# Autodesk Inventor assembly: ArmSquare
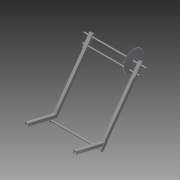
[picture p0: Inventor's stored thumbnail of the model, 180x180]
Saved by Autodesk Inventor 2013 (Build 170138000, 138)
## iProperties
Created: 2014-01-20
Part Number: ArmSquare
Document SubType Name: Assembly
Designer: RobertB
Author: RobertB
## Documents named in this file (10)
- E:\Robotics\FRC\2014\CAD\Robot\Catapult\Arm\ArmSquare.iam
- E:\Robotics\FRC\2014\CAD\Robot\Catapult\Arm\BarHolder.ipt
- E:\Robotics\FRC\2014\CAD\Robot\Catapult\Arm\CatapultAxle.ipt
- E:\Robotics\FRC\2014\CAD\Robot\Catapult\Arm\CatapultSprocket.ipt
- E:\Robotics\FRC\2014\CAD\Robot\Catapult\Arm\CatapultAxleSupportSquare.ipt
- E:\Robotics\FRC\2014\CAD\Robot\Catapult\Arm\SquareCrossBrace.ipt
- E:\Robotics\FRC\2014\CAD\Robot\Catapult\Arm\Imported Components\am-0077a-500 Key Hub r2\am-0077a-500 Key Hub r2.ipt
- E:\Robotics\FRC\2014\CAD\Robot\Catapult\Arm\CatapultArmSquare-Bottom.ipt
- E:\Robotics\FRC\2014\CAD\Robot\Catapult\Arm\CatapultArmSquare-Top.ipt
- E:\Robotics\FRC\2014\CAD\Robot\Catapult\Arm\CatapultArmSquare-Thickener.ipt
## Components (13 placed, 9 different names)
1. BarHolder:1 — Mate:19, Mate:36, Flush:15, Flush:16, Mate:38, Flush:18
2. BarHolder:2 — Mate:20, Flush:8, Flush:16, Flush:17, Mate:37, Mate:39
3. CatapultAxle:1 — Mate:4, Mate:17, Mate:30, Flush:14
4. CatapultSprocket:1 — Mate:4, Mate:16, Mate:18, Mate:32, Mate:34
5. SquareCrossBrace:1 — Mate:19, Mate:20, Flush:8, Mate:36, Flush:15
6. CatapultAxleSupportSquare:1 — Mate:34, Mate:35, Flush:13
7. Hub — Mate:16, Mate:17, Mate:18
8. CatapultArmSquare-Bottom:1 — Mate:21, Flush:9, Mate:22, Flush:12, Mate:39
9. CatapultArmSquare-Bottom:2 — Mate:23, Flush:10, Mate:24, Flush:12
10. CatapultArmSquare-Top:1 — Mate:21, Flush:9, Mate:22, Flush:11, Mate:25, Mate:26, Mate:27, Mate:31, Mate:32, Flush:17, Mate:37
11. CatapultArmSquare-Top:2 — Mate:23, Flush:10, Mate:24, Flush:11, Mate:28, Mate:29, Mate:31, Mate:33, Mate:38, Flush:18
12. CatapultArmSquare-Thickener:1 — Mate:28, Mate:29, Mate:33
13. CatapultArmSquare-Thickener:2 — Mate:25, Mate:26, Mate:27, Mate:30, Mate:35, Flush:13, Flush:14
## Relationships (36: Mate 25, Flush 11)
- Mate:4: CatapultAxle:1 ↔ CatapultSprocket:1
- Mate:16: CatapultSprocket:1 ↔ Hub
- Mate:17: CatapultAxle:1 ↔ Hub
- Mate:18: CatapultSprocket:1 ↔ Hub
- Mate:19: BarHolder:1 ↔ SquareCrossBrace:1
- Mate:20: BarHolder:2 ↔ SquareCrossBrace:1
- Flush:8: BarHolder:2 ↔ SquareCrossBrace:1
- Mate:21: CatapultArmSquare-Bottom:1 ↔ CatapultArmSquare-Top:1
- Flush:9: CatapultArmSquare-Bottom:1 ↔ CatapultArmSquare-Top:1
- Mate:22: CatapultArmSquare-Bottom:1 ↔ CatapultArmSquare-Top:1
- Mate:23: CatapultArmSquare-Bottom:2 ↔ CatapultArmSquare-Top:2
- Flush:10: CatapultArmSquare-Bottom:2 ↔ CatapultArmSquare-Top:2
- Mate:24: CatapultArmSquare-Bottom:2 ↔ CatapultArmSquare-Top:2
- Flush:11: CatapultArmSquare-Top:1 ↔ CatapultArmSquare-Top:2
- Flush:12: CatapultArmSquare-Bottom:1 ↔ CatapultArmSquare-Bottom:2
- Mate:25: CatapultArmSquare-Top:1 ↔ CatapultArmSquare-Thickener:2
- Mate:26: CatapultArmSquare-Top:1 ↔ CatapultArmSquare-Thickener:2
- Mate:27: CatapultArmSquare-Top:1 ↔ CatapultArmSquare-Thickener:2
- Mate:28: CatapultArmSquare-Top:2 ↔ CatapultArmSquare-Thickener:1
- Mate:29: CatapultArmSquare-Top:2 ↔ CatapultArmSquare-Thickener:1
- Mate:30: CatapultAxle:1 ↔ CatapultArmSquare-Thickener:2
- Mate:31 (406.4 mm): CatapultArmSquare-Top:1 ↔ CatapultArmSquare-Top:2
- Mate:32 (38.1 mm): CatapultSprocket:1 ↔ CatapultArmSquare-Top:1
- Mate:33: CatapultArmSquare-Top:2 ↔ CatapultArmSquare-Thickener:1
- Mate:34: CatapultSprocket:1 ↔ CatapultAxleSupportSquare:1
- Mate:35: CatapultAxleSupportSquare:1 ↔ CatapultArmSquare-Thickener:2
- Flush:13 (19.05 mm): CatapultAxleSupportSquare:1 ↔ CatapultArmSquare-Thickener:2
- Flush:14 (44.45 mm): CatapultAxle:1 ↔ CatapultArmSquare-Thickener:2
- Mate:36: BarHolder:1 ↔ SquareCrossBrace:1
- Flush:15: BarHolder:1 ↔ SquareCrossBrace:1
- Flush:16: BarHolder:1 ↔ BarHolder:2
- Flush:17: BarHolder:2 ↔ CatapultArmSquare-Top:1
- Mate:37: BarHolder:2 ↔ CatapultArmSquare-Top:1
- Mate:38: BarHolder:1 ↔ CatapultArmSquare-Top:2
- Flush:18: BarHolder:1 ↔ CatapultArmSquare-Top:2
- Mate:39 (-15.875 mm): BarHolder:2 ↔ CatapultArmSquare-Bottom:1
